# Autodesk Inventor assembly: Assembly4
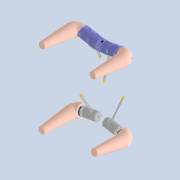
[picture p0: Inventor's stored thumbnail of the model, 180x180]
Saved by Autodesk Inventor 2020 (Build 240168000, 168)
## iProperties
Created: 2020-07-18
Part Number: Assembly4
Document SubType Name: Assembly
Designer: boxi
Author: boxi
## Documents named in this file (8)
- F:\soft robot\FlexipodHardware\mechanical_model\flexipod_ssembly.iam
- F:\soft robot\FlexipodHardware\mechanical_model\RoboMaster_M3508_Motor\RoboMaster M3508 P19 Brushless DC Gear Motor.iam
- F:\soft robot\FlexipodHardware\mechanical_model\bearing_30x42x7.ipt
- F:\soft robot\FlexipodHardware\mechanical_model\leg_coupler.ipt
- F:\soft robot\FlexipodHardware\mechanical_model\leg.ipt
- F:\soft robot\FlexipodHardware\mechanical_model\raspberry-pi-camera-module-v2-1\RspCameraMia.iam
- F:\soft robot\FlexipodHardware\mechanical_model\soft_body.ipt
- F:\soft robot\FlexipodHardware\mechanical_model\battery_6s_1550_ovonic.ipt
## Components (19 placed, 7 different names)
1. soft_body:1 — Rigid:1, Rigid:3, Rigid:4, Rigid:2, Mate:21, Angle:2, Mate:22, Mate:23, Mate:24
2. RoboMaster M3508 P19 Brushless DC Gear Motor:1 [sub-assembly] — Rigid:1, Mate:5, Mate:6, Mate:13, Rotational:5
3. RoboMaster M3508 P19 Brushless DC Gear Motor:2 [sub-assembly] — Rigid:3, Mate:7, Mate:8, Mate:16, Rotational:4
4. RoboMaster M3508 P19 Brushless DC Gear Motor:3 [sub-assembly] — Rigid:2, Mate:9, Mate:10, Mate:14, Rotational:6
5. RoboMaster M3508 P19 Brushless DC Gear Motor:4 [sub-assembly] — Rigid:4, Mate:11, Mate:15, Mate:17, Rotational:3
6. bearing_30x42x7:1 — Rotational:3
7. bearing_30x42x7:2 — Rotational:6
8. bearing_30x42x7:3 — Rotational:4
9. bearing_30x42x7:4 — Rotational:5
10. leg_coupler:1 — Mate:5, Mate:6, Rotational:11, Mate:13
11. leg_coupler:2 — Mate:9, Mate:10, Rotational:12, Mate:14
12. leg_coupler:3 — Mate:7, Mate:8, Rotational:14, Mate:16
13. leg_coupler:4 — Mate:11, Rotational:13, Mate:15, Mate:17
14. leg:1 — Rotational:11
15. leg:2 — Rotational:14
16. leg:3 — Rotational:12
17. leg:4 — Rotational:13
18. RspCameraMia:1 [sub-assembly] — Mate:22, Mate:23, Mate:24
19. battery_6s_1550_ovonic:1 — Mate:21, Angle:2
## Relationships (29: Mate 16, RevoluteJoint 8, WeldJoint 4, Angle 1)
- Rigid:1 [WeldJoint]: soft_body:1 ↔ RoboMaster M3508 P19 Brushless DC Gear Motor:1
- Rigid:3 [WeldJoint]: soft_body:1 ↔ RoboMaster M3508 P19 Brushless DC Gear Motor:2
- Rigid:4 [WeldJoint]: soft_body:1 ↔ RoboMaster M3508 P19 Brushless DC Gear Motor:4
- Rigid:2 [WeldJoint]: soft_body:1 ↔ RoboMaster M3508 P19 Brushless DC Gear Motor:3
- Rotational:3 [RevoluteJoint]: RoboMaster M3508 P19 Brushless DC Gear Motor:4 ↔ bearing_30x42x7:1
- Rotational:4 [RevoluteJoint]: RoboMaster M3508 P19 Brushless DC Gear Motor:2 ↔ bearing_30x42x7:3
- Rotational:5 [RevoluteJoint]: RoboMaster M3508 P19 Brushless DC Gear Motor:1 ↔ bearing_30x42x7:4
- Rotational:6 [RevoluteJoint]: RoboMaster M3508 P19 Brushless DC Gear Motor:3 ↔ bearing_30x42x7:2
- Mate:5 (0.1 mm): RoboMaster M3508 P19 Brushless DC Gear Motor:1 ↔ leg_coupler:1
- Mate:6: RoboMaster M3508 P19 Brushless DC Gear Motor:1 ↔ leg_coupler:1
- Mate:7 (0.1 mm): RoboMaster M3508 P19 Brushless DC Gear Motor:2 ↔ leg_coupler:3
- Mate:8: RoboMaster M3508 P19 Brushless DC Gear Motor:2 ↔ leg_coupler:3
- Mate:9 (0.1 mm): RoboMaster M3508 P19 Brushless DC Gear Motor:3 ↔ leg_coupler:2
- Mate:10: RoboMaster M3508 P19 Brushless DC Gear Motor:3 ↔ leg_coupler:2
- Mate:11 (0.1 mm): RoboMaster M3508 P19 Brushless DC Gear Motor:4 ↔ leg_coupler:4
- Rotational:11 [RevoluteJoint]: leg_coupler:1 ↔ leg:1
- Rotational:12 [RevoluteJoint]: leg_coupler:2 ↔ leg:3
- Rotational:13 [RevoluteJoint]: leg_coupler:4 ↔ leg:4
- Rotational:14 [RevoluteJoint]: leg_coupler:3 ↔ leg:2
- Mate:13: RoboMaster M3508 P19 Brushless DC Gear Motor:1 ↔ leg_coupler:1
- Mate:14: RoboMaster M3508 P19 Brushless DC Gear Motor:3 ↔ leg_coupler:2
- Mate:15: RoboMaster M3508 P19 Brushless DC Gear Motor:4 ↔ leg_coupler:4
- Mate:16: RoboMaster M3508 P19 Brushless DC Gear Motor:2 ↔ leg_coupler:3
- Mate:17: RoboMaster M3508 P19 Brushless DC Gear Motor:4 ↔ leg_coupler:4
- Mate:21: soft_body:1 ↔ battery_6s_1550_ovonic:1
- Angle:2 (0 deg): soft_body:1 ↔ battery_6s_1550_ovonic:1
- Mate:22: soft_body:1 ↔ RspCameraMia:1
- Mate:23: soft_body:1 ↔ RspCameraMia:1
- Mate:24: soft_body:1 ↔ RspCameraMia:1
## Named parameters: motor_adaptor_offset = 0.1 mm
